# Autodesk Inventor assembly: Baugruppe Fuß
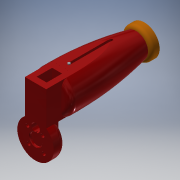
[picture p0: Inventor's stored thumbnail of the model, 180x180]
Saved by Autodesk Inventor 2019 (Build 230136000, 136)
## iProperties
Created: 2018-07-23
Part Number: Baugruppe Fuß
Material: Generisch
Document SubType Name: Assembly
Designer: 1eule14
Author: 1eule14
## Documents named in this file (4)
- H:\Eule\Bauteile\Fuß\Baugruppe Fuß.iam
- H:\Eule\Bauteile\Fuß\Fuß.ipt
- H:\Eule\Bauteile\Fuß\Stift.ipt
- H:\Eule\Bauteile\Fuß\Motorhalterung.ipt
## Components (3 placed, 3 different names)
1. Fuß:1 — Fluchtend:1, Passend:1, Passend:2, Passend:3
2. Stift:1 — Passend:1
3. Motorhalterung:1 — Passend:2, Passend:3
## Relationships (4: Mate 3, Flush 1)
- Fluchtend:1 [Flush]: Fuß:1
- Passend:1 [Mate]: Fuß:1 ↔ Stift:1
- Passend:2 [Mate]: Fuß:1 ↔ Motorhalterung:1
- Passend:3 [Mate]: Fuß:1 ↔ Motorhalterung:1
